# Autodesk Inventor assembly: Bio
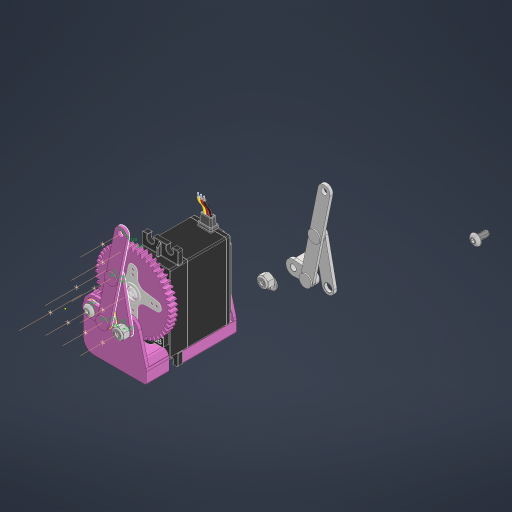
[picture p0: Inventor's stored thumbnail of the model, 512x512]
Saved by Autodesk Inventor 2024.1 (Build 281209000, 209)
## iProperties
Created: 2023-11-14
Part Number: Bio
Document SubType Name: Assembly
Designer: Brandon
Author: Brandon
## Documents named in this file (11)
- C:\Users\Brandon\Documents\School\FallCAD\Bio\Bio.iam
- C:\Users\Brandon\Documents\School\FallCAD\Bio\Servo HS425BB\Servo HS425BB.ipt
- C:\Users\Brandon\Documents\School\FallCAD\Bio\Bio\Design Accelerator\Spur Gears1.iam
- C:\Users\Brandon\Documents\School\FallCAD\Bio\Bio50t.ipt
- C:\Users\Brandon\Documents\School\FallCAD\Bio\Alignment.ipt
- C:\Users\Brandon\Documents\School\FallCAD\Bio\Bio12tNew.ipt
- C:\Users\Brandon\Documents\School\FallCAD\Bio\ServoMount.ipt
- C:\Users\Brandon\Documents\School\FallCAD\Bio\FrontLinkage.ipt
- C:\Users\Brandon\Documents\School\FallCAD\Bio\92095A179_Button Head Hex Drive Screw\92095A179_Button Head Hex Drive Screw.ipt
- C:\Users\Brandon\Documents\School\FallCAD\Bio\M3Spacer.ipt
- C:\Users\Brandon\Documents\School\FallCAD\Bio\90576A102_Medium-Strength Steel Nylon-Insert Locknut\90576A102_Medium-Strength Steel Nylon-Insert Locknut.ipt
## Components (16 placed, 10 different names)
1. Servo HS425BB:1 — Flush:1
2. Bio50t:1 — Mate:1, Flush:1, Flush:2
3. Alignment:1 — Mate:1, Mate:2
4. Spur Gears:1 [sub-assembly]
5. Bio12tNew:1 — Mate:2, Flush:2, Flush:3, Mate:3, Insert:1
6. ServoMount:1 — Insert:2, Insert:5
7. FrontLinkage:1 — Mate:3, Insert:1, Insert:3, Insert:4
8. 92095A179_Button Head Hex Drive Screw:1 — Insert:2
9. M3Spacer:1
10. 90576A102_Medium-Strength Steel Nylon-Insert Locknut:1 — Insert:3
11. 92095A179_Button Head Hex Drive Screw:2 — Insert:4
12. 92095A179_Button Head Hex Drive Screw:3 — Insert:5
13. 90576A102_Medium-Strength Steel Nylon-Insert Locknut:2
14. FrontLinkage:2
15. 92095A179_Button Head Hex Drive Screw:4
16. M3Spacer:2
## Relationships (11: Insert 5, Mate 3, Flush 3)
- Mate:1: Bio50t:1 ↔ Alignment:1
- Flush:1: Servo HS425BB:1 ↔ Bio50t:1
- Mate:2: Alignment:1 ↔ Bio12tNew:1
- Flush:2 (-0.762 mm): Bio50t:1 ↔ Bio12tNew:1
- Flush:3 (0.127 mm): Bio12tNew:1
- Mate:3: Bio12tNew:1 ↔ FrontLinkage:1
- Insert:1: Bio12tNew:1 ↔ FrontLinkage:1
- Insert:2: ServoMount:1 ↔ 92095A179_Button Head Hex Drive Screw:1
- Insert:3: FrontLinkage:1 ↔ 90576A102_Medium-Strength Steel Nylon-Insert Locknut:1
- Insert:4: FrontLinkage:1 ↔ 92095A179_Button Head Hex Drive Screw:2
- Insert:5: ServoMount:1 ↔ 92095A179_Button Head Hex Drive Screw:3
